# Autodesk Inventor assembly: completo
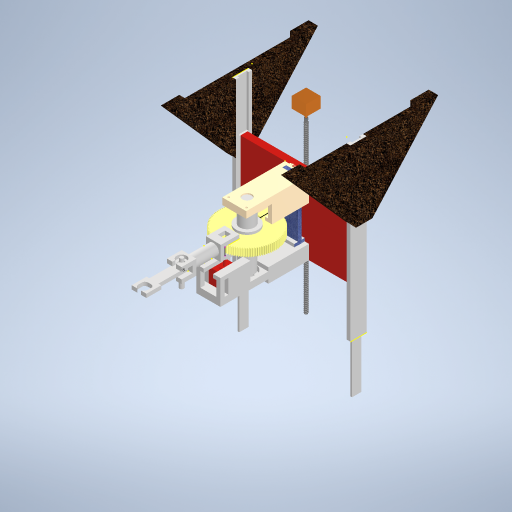
[picture p0: Inventor's stored thumbnail of the model, 512x512]
Saved by Autodesk Inventor 2023 (Build 270158000, 158)
## iProperties
Created: 2023-03-27
Part Number: completo
Document SubType Name: Assembly
Designer: sebas
Author: sebas
## Documents named in this file (11)
- E:\Unlz\PROYECTO FINAL\recibida\completo.iam
- E:\Unlz\PROYECTO FINAL\version final\escuadra.ipt
- E:\Unlz\PROYECTO FINAL\version final\GUIA INTERIOR.ipt
- E:\Unlz\PROYECTO FINAL\version final\Part1.ipt
- E:\Unlz\PROYECTO FINAL\version final\base vertical.ipt
- E:\Unlz\PROYECTO FINAL\version final\base horiz.ipt
- E:\Unlz\PROYECTO FINAL\version final\sin fin.ipt
- E:\Unlz\PROYECTO FINAL\version final\BRAZO22.ipt
- E:\Unlz\PROYECTO FINAL\version final\MOTOR.ipt
- E:\Unlz\PROYECTO FINAL\version final\agarre sin fin.ipt
- E:\Unlz\PROYECTO FINAL\recibida\ensamble.iam
## Components (13 placed, 10 different names)
1. escuadra:1 — Mate:3, Mate:4, Flush:3, Flush:6, Flush:37
2. escuadra:2 — Mate:5, Mate:6, Flush:4, Flush:6, Flush:31, Flush:35
3. GUIA INTERIOR:1 — Mate:7, Mate:8, Flush:5, Mate:9, Flush:7, Flush:8
4. GUIA INTERIOR:2 — Mate:1, Mate:2, Flush:5, Mate:10
5. Part1:1 — Flush:2, Mate:5, Mate:6, Flush:4, Mate:7, Mate:8, Flush:32
6. Part1:2 — Mate:1, Mate:2, Flush:2, Mate:3, Mate:4, Flush:3
7. base vertical:1 — Mate:9, Mate:10, Flush:7, Mate:12, Flush:8, Flush:9, Flush:10, Mate:31, Flush:33, Flush:35, Flush:36, Mate:33
8. base horiz:1 — Mate:12, Flush:9, Flush:10
9. sin fin:1 — Mate:24, Mate:25, Mate:30
10. BRAZO22:1
11. MOTOR:1 — Mate:24, Mate:25, Flush:31
12. agarre sin fin:1 — Mate:30, Mate:31, Flush:32, Flush:33
13. ensamble:1 [sub-assembly] — Flush:36, Mate:33, Flush:37
## Relationships (31: Mate 16, Flush 15)
- Mate:1: GUIA INTERIOR:2 ↔ Part1:2
- Mate:2: GUIA INTERIOR:2 ↔ Part1:2
- Flush:2: Part1:1 ↔ Part1:2
- Mate:3: escuadra:1 ↔ Part1:2
- Mate:4: escuadra:1 ↔ Part1:2
- Flush:3: escuadra:1 ↔ Part1:2
- Mate:5: escuadra:2 ↔ Part1:1
- Mate:6: escuadra:2 ↔ Part1:1
- Flush:4: escuadra:2 ↔ Part1:1
- Mate:7: GUIA INTERIOR:1 ↔ Part1:1
- Mate:8: GUIA INTERIOR:1 ↔ Part1:1
- Flush:5: GUIA INTERIOR:1 ↔ GUIA INTERIOR:2
- Flush:6: escuadra:1 ↔ escuadra:2
- Mate:9: GUIA INTERIOR:1 ↔ base vertical:1
- Mate:10: GUIA INTERIOR:2 ↔ base vertical:1
- Flush:7 (260 mm): GUIA INTERIOR:1 ↔ base vertical:1
- Mate:12: base vertical:1 ↔ base horiz:1
- Flush:8 (2.975 mm): GUIA INTERIOR:1 ↔ base vertical:1
- Flush:9 (167.3 mm): base vertical:1 ↔ base horiz:1
- Flush:10 (25 mm): base vertical:1 ↔ base horiz:1
- Mate:24: sin fin:1 ↔ MOTOR:1
- Mate:25: sin fin:1 ↔ MOTOR:1
- Flush:31: escuadra:2 ↔ MOTOR:1
- Mate:30: sin fin:1 ↔ agarre sin fin:1
- Mate:31: base vertical:1 ↔ agarre sin fin:1
- Flush:32 (165 mm): Part1:1 ↔ agarre sin fin:1
- Flush:33 (80 mm): base vertical:1 ↔ agarre sin fin:1
- Flush:35 (194.0052 mm): escuadra:2 ↔ base vertical:1
- Flush:36: base vertical:1 ↔ ensamble:1
- Mate:33: base vertical:1 ↔ ensamble:1
- Flush:37 (140 mm): escuadra:1 ↔ ensamble:1
